# Autodesk Inventor assembly: ROBAL_2.0_assembly_01
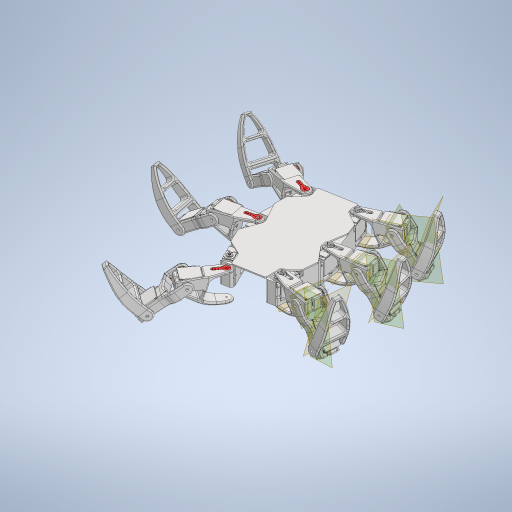
[picture p0: Inventor's stored thumbnail of the model, 512x512]
Saved by Autodesk Inventor 2023.4 (Build 274418000, 418)
## iProperties
Created: 2024-06-29
Part Number: ROBAL_2.0_assembly_01
Document SubType Name: Assembly
Designer: kamil
Author: kamil
## Documents named in this file (14)
- E:\PROJECTS_REPOS\Robal-2.0\mechanics\ROBAL_2.0_assembly_01.iam
- E:\PROJECTS_REPOS\Robal-2.0\mechanics\Standard-Servo.ipt
- E:\PROJECTS_REPOS\Robal-2.0\mechanics\gora.ipt
- E:\PROJECTS_REPOS\Robal-2.0\mechanics\noga_pre.iam
- E:\PROJECTS_REPOS\Robal-2.0\mechanics\Standard-Servo_MIR3.ipt
- E:\PROJECTS_REPOS\Robal-2.0\mechanics\dol.ipt
- C:\Users\kamil\Documents\PROJECTS - repos\Robal---Hexapod\mechanics\Raspberry Pi 4 Model B.ipt
- E:\PROJECTS_REPOS\Robal-2.0\mechanics\noga_pre_MIR1.iam
- E:\PROJECTS_REPOS\Robal-2.0\mechanics\uchwyt_serwa_podwojny.ipt
- E:\PROJECTS_REPOS\Robal-2.0\mechanics\uchwyt_serwa_podwojny_MIR.ipt
- E:\PROJECTS_REPOS\Robal-2.0\mechanics\DC-DC Step Down Buck Converter CC-CV 300W 9A.ipt
- E:\PROJECTS_REPOS\Robal-2.0\mechanics\Bashing_3S1P_11.1V_5000mAH_60c.ipt
- E:\PROJECTS_REPOS\Robal-2.0\mechanics\Lithium Battery Capacity Indicator Module.ipt
- E:\PROJECTS_REPOS\Robal-2.0\mechanics\XL4015_MODELO_PISTAS.ipt
## Components (22 placed, 13 different names)
1. Standard-Servo:1 — Zestawiające:5, Zestawiające:63, Zestawiające:64, Zestawiające:65, Zestawiające:66
2. gora:1 — Zestawiające:5, Zestawiające:10, Zestawiające:19, Zestawiające:35, Zestawiające:41, Zestawiające:42, Równoległe:4, Zestawiające:46, Zestawiające:47, Zestawiające:51, Równoległe:5, Zestawiające:61, Zestawiające:72
3. Standard-Servo:2 — Zestawiające:10, Zestawiające:53, Zestawiające:54
4. noga_pre:3 [sub-assembly] — Zestawiające:19, Zestawiające:63, Zestawiające:64
5. Standard-Servo_MIR3:1 — Zestawiające:59, Zestawiające:61, Zestawiające:62, Zestawiające:67, Zestawiające:68
6. Standard-Servo_MIR3:2 — Zestawiające:47, Zestawiające:48, Zestawiające:49, Zestawiające:55, Zestawiające:56
7. Standard-Servo:3 — Zestawiające:35, Zestawiające:50, Zestawiające:52
8. Standard-Servo:4 — Zestawiające:43, Zestawiające:44, Zestawiające:45, Zestawiające:46
9. dol:1 — Zestawiające:70, Zestawiające:71, Kątowe:2
10. noga_pre:4 [sub-assembly]
11. noga_pre:5 [sub-assembly]
12. Raspberry Pi 4 Model B:1 — Zestawiające:41
13. noga_pre_MIR1:1 [sub-assembly] — Zestawiające:59, Zestawiające:62
14. noga_pre_MIR1:2 [sub-assembly]
15. noga_pre_MIR1:3 [sub-assembly] — Zestawiające:55, Zestawiające:56
16. uchwyt_serwa_podwojny:1 — Zestawiające:42, Równoległe:4, Zestawiające:43, Zestawiające:44, Zestawiające:45, Zestawiające:48, Zestawiające:49, Równoległe:6, Zestawiające:67, Zestawiające:68, Kątowe:1
17. uchwyt_serwa_podwojny_MIR:1 — Zestawiające:50, Zestawiające:51, Równoległe:5, Równoległe:6, Zestawiające:52, Zestawiające:53, Zestawiające:54, Zestawiające:65, Zestawiające:66, Równoległe:9
18. DC-DC Step Down Buck Converter CC-CV 300W 9A:1 — Równoległe:7, Równoległe:8, Zestawiające:69, Zestawiające:70, Kątowe:1
19. DC-DC Step Down Buck Converter CC-CV 300W 9A:2 — Równoległe:7, Równoległe:8, Zestawiające:69
20. Bashing_3S1P_11.1V_5000mAH_60c:1 — Zestawiające:71, Kątowe:2
21. Lithium Battery Capacity Indicator Module:1 — Równoległe:9, Zestawiające:72
22. XL4015_MODELO_PISTAS:1
## Relationships (41: Mate 33, Flush 6, Angle 2)
- Zestawiające:5 [Mate]: Standard-Servo:1 ↔ gora:1
- Zestawiające:10 [Mate]: gora:1 ↔ Standard-Servo:2
- Zestawiające:19 [Mate]: gora:1 ↔ noga_pre:3
- Zestawiające:35 [Mate]: gora:1 ↔ Standard-Servo:3
- Zestawiające:41 [Mate]: gora:1 ↔ Raspberry Pi 4 Model B:1
- Zestawiające:42 [Mate]: gora:1 ↔ uchwyt_serwa_podwojny:1
- Równoległe:4 [Flush]: gora:1 ↔ uchwyt_serwa_podwojny:1
- Zestawiające:43 [Mate] (1 mm): Standard-Servo:4 ↔ uchwyt_serwa_podwojny:1
- Zestawiające:44 [Mate]: Standard-Servo:4 ↔ uchwyt_serwa_podwojny:1
- Zestawiające:45 [Mate] (1 mm): Standard-Servo:4 ↔ uchwyt_serwa_podwojny:1
- Zestawiające:46 [Mate]: gora:1 ↔ Standard-Servo:4
- Zestawiające:47 [Mate]: gora:1 ↔ Standard-Servo_MIR3:2
- Zestawiające:48 [Mate]: Standard-Servo_MIR3:2 ↔ uchwyt_serwa_podwojny:1
- Zestawiające:49 [Mate] (1 mm): Standard-Servo_MIR3:2 ↔ uchwyt_serwa_podwojny:1
- Zestawiające:50 [Mate]: Standard-Servo:3 ↔ uchwyt_serwa_podwojny_MIR:1
- Zestawiające:51 [Mate]: gora:1 ↔ uchwyt_serwa_podwojny_MIR:1
- Równoległe:5 [Flush]: gora:1 ↔ uchwyt_serwa_podwojny_MIR:1
- Równoległe:6 [Flush]: uchwyt_serwa_podwojny:1 ↔ uchwyt_serwa_podwojny_MIR:1
- Zestawiające:52 [Mate] (1 mm): Standard-Servo:3 ↔ uchwyt_serwa_podwojny_MIR:1
- Zestawiające:53 [Mate]: Standard-Servo:2 ↔ uchwyt_serwa_podwojny_MIR:1
- Zestawiające:54 [Mate] (1 mm): Standard-Servo:2 ↔ uchwyt_serwa_podwojny_MIR:1
- Zestawiające:55 [Mate] (2.1 mm): Standard-Servo_MIR3:2 ↔ noga_pre_MIR1:3
- Zestawiające:56 [Mate]: Standard-Servo_MIR3:2 ↔ noga_pre_MIR1:3
- Zestawiające:59 [Mate] (2.1 mm): Standard-Servo_MIR3:1 ↔ noga_pre_MIR1:1
- Zestawiające:61 [Mate]: gora:1 ↔ Standard-Servo_MIR3:1
- Zestawiające:62 [Mate]: Standard-Servo_MIR3:1 ↔ noga_pre_MIR1:1
- Zestawiające:63 [Mate]: Standard-Servo:1 ↔ noga_pre:3
- Zestawiające:64 [Mate] (2.1 mm): Standard-Servo:1 ↔ noga_pre:3
- Zestawiające:65 [Mate]: Standard-Servo:1 ↔ uchwyt_serwa_podwojny_MIR:1
- Zestawiające:66 [Mate] (1 mm): Standard-Servo:1 ↔ uchwyt_serwa_podwojny_MIR:1
- Zestawiające:67 [Mate]: Standard-Servo_MIR3:1 ↔ uchwyt_serwa_podwojny:1
- Zestawiające:68 [Mate] (1 mm): Standard-Servo_MIR3:1 ↔ uchwyt_serwa_podwojny:1
- Równoległe:7 [Flush]: DC-DC Step Down Buck Converter CC-CV 300W 9A:1 ↔ DC-DC Step Down Buck Converter CC-CV 300W 9A:2
- Równoległe:8 [Flush]: DC-DC Step Down Buck Converter CC-CV 300W 9A:1 ↔ DC-DC Step Down Buck Converter CC-CV 300W 9A:2
- Zestawiające:69 [Mate] (-22 mm): DC-DC Step Down Buck Converter CC-CV 300W 9A:1 ↔ DC-DC Step Down Buck Converter CC-CV 300W 9A:2
- Zestawiające:70 [Mate] (3 mm): dol:1 ↔ DC-DC Step Down Buck Converter CC-CV 300W 9A:1
- Kątowe:1 [Angle] (0 deg): uchwyt_serwa_podwojny:1 ↔ DC-DC Step Down Buck Converter CC-CV 300W 9A:1
- Zestawiające:71 [Mate]: dol:1 ↔ Bashing_3S1P_11.1V_5000mAH_60c:1
- Kątowe:2 [Angle] (0 deg): dol:1 ↔ Bashing_3S1P_11.1V_5000mAH_60c:1
- Równoległe:9 [Flush]: uchwyt_serwa_podwojny_MIR:1 ↔ Lithium Battery Capacity Indicator Module:1
- Zestawiające:72 [Mate]: gora:1 ↔ Lithium Battery Capacity Indicator Module:1
